# Autodesk Inventor assembly: Skirt Front [A]
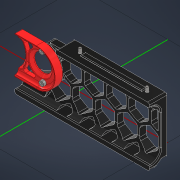
[picture p0: Inventor's stored thumbnail of the model, 180x180]
Saved by Autodesk Inventor 2022 (Build 260153000, 153)
## iProperties
Created: 2022-03-13
Part Number: Skirt Front [A]
Document SubType Name: Assembly
Designer: sleib
Author: sleib
## Documents named in this file (5)
- C:\Users\sleib\Projekte\Voron-2\CAD\Inventor\Skirt Front [A].iam
- C:\Users\sleib\Projekte\Voron-2\CAD\Inventor\Skirt Front (350mm) [A].ipt
- C:\Users\sleib\Projekte\Voron-2\CAD\Inventor\Skirt Belt-Guard.ipt
- C:\Users\sleib\Projekte\Voron-2\CAD\Inventor\M3 Threaded Insert.ipt
- C:\Users\sleib\Projekte\Voron-2\CAD\Inventor\M3x8 SHCS.ipt
## Components (9 placed, 4 different names)
1. Skirt Front (350mm) [A]:1 — Passend:1, Passend:2, Fluchtend:1, Fluchtend:2, Passend:3, Fluchtend:3, Passend:10, Passend:11, Passend:12, Passend:13, Passend:14
2. Skirt Belt-Guard:1 — Passend:4, Passend:5, Passend:6, Passend:7, Passend:10
3. M3 Threaded Insert:1 — Passend:1, Fluchtend:1, Passend:8
4. M3 Threaded Insert:2 — Passend:2, Fluchtend:2, Passend:9
5. M3 Threaded Insert:3 — Passend:3, Fluchtend:3
6. M3x8 SHCS:1 — Passend:4, Passend:7, Passend:8
7. M3x8 SHCS:2 — Passend:5, Passend:6, Passend:9
8. M3x8 SHCS:3 — Passend:11, Passend:13
9. M3x8 SHCS:4 — Passend:12, Passend:14
## Relationships (17: Mate 14, Flush 3)
- Passend:1 [Mate]: Skirt Front (350mm) [A]:1 ↔ M3 Threaded Insert:1
- Passend:2 [Mate]: Skirt Front (350mm) [A]:1 ↔ M3 Threaded Insert:2
- Fluchtend:1 [Flush]: Skirt Front (350mm) [A]:1 ↔ M3 Threaded Insert:1
- Fluchtend:2 [Flush]: Skirt Front (350mm) [A]:1 ↔ M3 Threaded Insert:2
- Passend:3 [Mate]: Skirt Front (350mm) [A]:1 ↔ M3 Threaded Insert:3
- Fluchtend:3 [Flush]: Skirt Front (350mm) [A]:1 ↔ M3 Threaded Insert:3
- Passend:4 [Mate]: Skirt Belt-Guard:1 ↔ M3x8 SHCS:1
- Passend:5 [Mate]: Skirt Belt-Guard:1 ↔ M3x8 SHCS:2
- Passend:6 [Mate]: Skirt Belt-Guard:1 ↔ M3x8 SHCS:2
- Passend:7 [Mate]: Skirt Belt-Guard:1 ↔ M3x8 SHCS:1
- Passend:8 [Mate]: M3 Threaded Insert:1 ↔ M3x8 SHCS:1
- Passend:9 [Mate]: M3 Threaded Insert:2 ↔ M3x8 SHCS:2
- Passend:10 [Mate]: Skirt Front (350mm) [A]:1 ↔ Skirt Belt-Guard:1
- Passend:11 [Mate]: Skirt Front (350mm) [A]:1 ↔ M3x8 SHCS:3
- Passend:12 [Mate]: Skirt Front (350mm) [A]:1 ↔ M3x8 SHCS:4
- Passend:13 [Mate]: Skirt Front (350mm) [A]:1 ↔ M3x8 SHCS:3
- Passend:14 [Mate]: Skirt Front (350mm) [A]:1 ↔ M3x8 SHCS:4
